# Autodesk Inventor assembly: ensemble_moteur_MIR
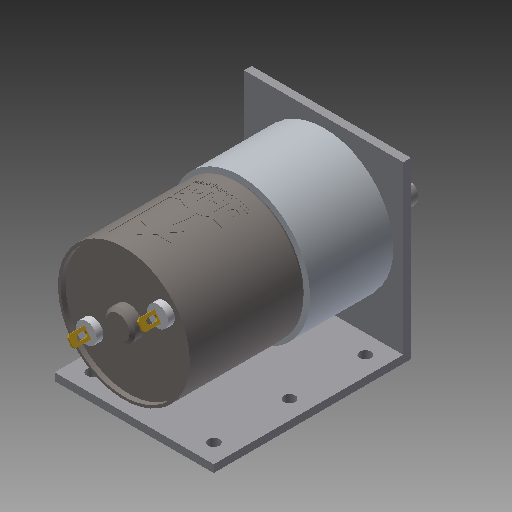
[picture p0: Inventor's stored thumbnail of the model, 512x512]
Saved by Autodesk Inventor 2017 (Build 210142000, 142)
## iProperties
Created: 2016-12-04
Part Number: ensemble_moteur_MIR
Document SubType Name: Assembly
Designer: Aegir
Author: Aegir
## Documents named in this file (3)
- C:\Users\franc\Desktop\EsialRobotik\Mecanique\base roulante_v2\conception\ensemble_moteur_MIR.iam
- C:\Users\franc\Desktop\EsialRobotik\Mecanique\base roulante_v2\conception\moteur\37d-gearmotor-19-30_MIR.ipt
- C:\Users\franc\Desktop\EsialRobotik\Mecanique\base roulante_v2\conception\support_moteur_MIR.ipt
## Components (2 placed, 2 different names)
1. 37d-gearmotor-19-30_MIR:1 — Affleurement:1
2. support_moteur_MIR:1 — Affleurement:1
## Relationships (1: Mate 1)
- Affleurement:1 [Mate]: 37d-gearmotor-19-30_MIR:1 ↔ support_moteur_MIR:1
